# Autodesk Inventor assembly: HHPMGS5
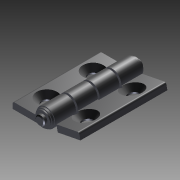
[picture p0: Inventor's stored thumbnail of the model, 180x180]
Saved by Autodesk Inventor 2015 SP1 (Build 190203100, 203)
## iProperties
Category: PARTsolutions
Company: MISUMI
Created: 2015-01-26
Part Number: HHPMGS5
Catalog Web Link: www.cadenas.de
Description: HHPMGS-Low Dust Raise Hinges
Vendor: MISUMI
Document SubType Name: Assembly
Designer: PARTuser1
Manufacturer: MISUMI
PSOL_IDENT_0: {\\10.0.0.236\data_v8\23d-libs\misumi\metric\39_accessories_for_al_extrusions\hhpmgs_asmtab.prj},165
PSOL_IDENT_1: {VTYP=3D},{STYP=ASSTAB},{NB=HHPMGS5},{LINA=HHPMGS5},{NN=HHPMGS},{DATE=17.11.2014 05:31:02},{GEOMDAT
PSOL_IDENT_2: E=18.12.2009},{VERSION=},{LINEID=10},{LINESUBID=-1},{WBVAR=ALT1}  {NB=HHPMGS5},{LINA=HHPMGS5},{KT=DU
PSOL_IDENT_3: MMY},{PN=HHPMGS5},{TYPE=HHPMGS},{MAT=6063S-T5 Aluminum Alloy},{MATB=Oil Soaked Polyacetal},{ST=Elect
PSOL_IDENT_4: roless Nickel Plating},{NO=5},{ALKG=10},{ALN=98},{MASS=22},{L=47},{W=36},{K=11.0},{P=25},{J=7.5},{S=
PSOL_IDENT_5: 21},{ND=5.5},{NC=11},{T=3.5},{E=5.0},{R=5.0},{AB=SHFBS5-8},{ABQ=4},{AN=HNTTSN5-5},{ANQ=4},{ALT1=},{A
PSOL_IDENT_6: BM=5},{ABL=8},{ANNO=5},{ANM=5},{PPATH=hhpmgs_asmtpl.prj}
SUPPLIER: MISUMI
ARTICLENO: HHPMGS5
BOMINFO: HHPMGS5
CREATOR: CADENAS GmbH
Title: HHPMGS5
Author: Cadenas PARTsolutions
Comments: Low Dust Raise Hinges
## Documents named in this file (4)
- C:\Users\Jack\ownCloud\Projects\CoreXY\InventorModel\Hardware\Hinges\HingeHHPMGS5\HHPMGS5.iam
- C:\Users\Jack\ownCloud\Projects\CoreXY\InventorModel\Hardware\Hinges\HingeHHPMGS5\HHPMGS5p1.ipt
- C:\Users\Jack\ownCloud\Projects\CoreXY\InventorModel\Hardware\Hinges\HingeHHPMGS5\HHPMGS5pin.ipt
- C:\Users\Jack\ownCloud\Projects\CoreXY\InventorModel\Hardware\Hinges\HingeHHPMGS5\HHPMGS5p2.ipt
## Components (3 placed, 3 different names)
1. HHPMGS5p1:1 — Mate:2
2. HHPMGS5pin:1 — Mate:1
3. HHPMGS5p2:1 — Mate:1, Mate:2
## Relationships (2: Mate 2)
- Mate:1: HHPMGS5pin:1 ↔ HHPMGS5p2:1
- Mate:2 (1 mm): HHPMGS5p1:1 ↔ HHPMGS5p2:1
